# Autodesk Inventor assembly: SAR330  x 5 + couplers right
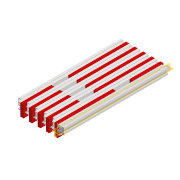
[picture p0: Inventor's stored thumbnail of the model, 180x180]
Saved by Autodesk Inventor 2020 (Build 240168000, 168)
## iProperties
Created: 2019-12-12
Part Number: SAR330  x 5 + couplers right
Document SubType Name: Assembly
Designer: ball
Author: ball
## Documents named in this file (3)
- C:\FTC\FTC8863CAD\2019 Robot\Delivery\Lift Right\SAR330  x 5 + couplers right.iam
- C:\FTC\FTC8863CAD\2019 Robot\Delivery\Lift Right\SAR330 x 4 + regular couplers right offset.iam
- C:\FTC\FTC8863CAD\2019 Robot\Delivery\Lift Right\SAR330 + fixed couplers right.iam
## Components (2 placed, 2 different names)
1. Assembly2:1 [sub-assembly] — Mate:1, Mate:2, Mate:3
2. SAR330 + fixed couplers right:1 [sub-assembly] — Mate:1, Mate:2, Mate:3
## Relationships (3: Mate 3)
- Mate:1: Assembly2:1 ↔ SAR330 + fixed couplers right:1
- Mate:2: Assembly2:1 ↔ SAR330 + fixed couplers right:1
- Mate:3: Assembly2:1 ↔ SAR330 + fixed couplers right:1
